# Autodesk Inventor assembly: Assy_all
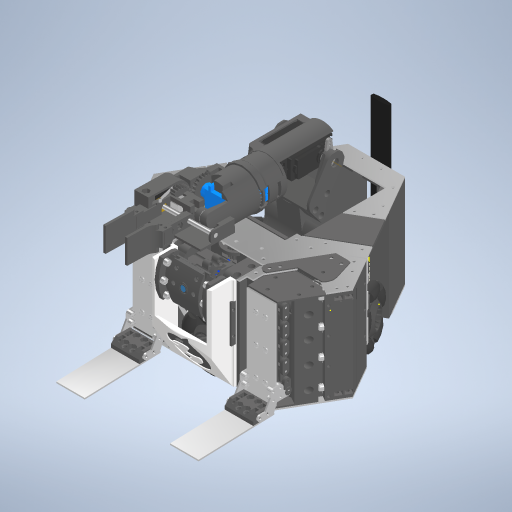
[picture p0: Inventor's stored thumbnail of the model, 512x512]
Saved by Autodesk Inventor 2024.1 (Build 281209000, 209)
## iProperties
Created: 2025-03-04
Part Number: Assy_all
Document SubType Name: Assembly
Designer: hibik
Author: hibik
## Documents named in this file (15)
- C:\Users\hibik\Documents\Robomech\RESCUE\ORCA\hard\Assy_all.iam
- C:\Users\hibik\Documents\Robomech\RESCUE\ORCA\hard\Assy_cam_connection.iam
- C:\Users\hibik\Documents\Robomech\RESCUE\ORCA\hard\flame_back\flame_back.ipt
- C:\Users\hibik\Documents\Robomech\RESCUE\ORCA\hard\board\core_power.iam
- C:\Users\hibik\Documents\Robomech\RESCUE\ORCA\hard\board\core_usp.iam
- C:\Users\hibik\Documents\Robomech\RESCUE\ORCA\hard\std_parts\battery.ipt
- C:\Users\hibik\Documents\Robomech\RESCUE\ORCA\hard\std_parts\emergency_button.ipt
- C:\Users\hibik\Documents\Robomech\RESCUE\ORCA\hard\flame_back\flame_upper_back.ipt
- C:\Users\hibik\Documents\Robomech\RESCUE\ORCA\hard\flame_back\flame_side_right.ipt
- C:\Users\hibik\Documents\Robomech\RESCUE\ORCA\hard\flame_back\flame_side_left.ipt
- C:\Users\hibik\Documents\Robomech\RESCUE\ORCA\hard\flame_back\battery_holder_spring.ipt
- C:\Users\hibik\Documents\Robomech\RESCUE\ORCA\hard\flame_back\battery_holder_cover.ipt
- C:\Users\hibik\Documents\Robomech\RESCUE\ORCA\hard\std_parts\Buffalo_Wl-U2-433DHP.ipt
- C:\Users\hibik\Documents\Robomech\RESCUE\ORCA\hard\flame_back\cover_setter_side_front.ipt
- C:\Users\hibik\Documents\Robomech\RESCUE\ORCA\hard\cover\Assy_cover_front.iam
## Components (15 placed, 14 different names)
1. Assy_cam_connection:1 [sub-assembly] — メイト:1, フラッシュ:1, フラッシュ:2, メイト:4, メイト:11, 挿入:7, 挿入:8, 挿入:9, 挿入:10, メイト:13, フラッシュ:10, メイト:14
2. flame_back:1 — メイト:1, フラッシュ:1, フラッシュ:2, 挿入:2, 挿入:3, メイト:2, フラッシュ:3, フラッシュ:4, メイト:5, メイト:6, メイト:8, フラッシュ:9, メイト:9, メイト:10, メイト:12
3. core_power:1 [sub-assembly] — 挿入:2, 挿入:3
4. battery:1 — メイト:10, メイト:11, メイト:12
5. core_usp:1 [sub-assembly] — 挿入:4, 挿入:5
6. emergency_button:1 — 挿入:6, 角度:1
7. flame_upper_back:1 — メイト:2, フラッシュ:3, フラッシュ:4, フラッシュ:5, フラッシュ:6, メイト:3, フラッシュ:7, フラッシュ:8, メイト:7
8. flame_side_right:1 — フラッシュ:5, フラッシュ:6, メイト:3, 挿入:4, 挿入:5
9. flame_side_left:1 — フラッシュ:7, フラッシュ:8, メイト:4, 挿入:6, 角度:1
10. battery_holder_spring:1 — メイト:5, メイト:6, メイト:7
11. battery_holder_cover:1 — メイト:8, フラッシュ:9, メイト:9
12. Buffalo_Wl-U2-433DHP:1
13. cover_setter_side_front:1 — 挿入:7, 挿入:8
14. cover_setter_side_front:2 — 挿入:9, 挿入:10
15. Assy_cover_front:1 [sub-assembly] — メイト:13, フラッシュ:10, メイト:14
## Relationships (34: Mate 14, Flush 10, Insert 9, Angle 1)
- メイト:1 [Mate]: Assy_cam_connection:1 ↔ flame_back:1
- フラッシュ:1 [Flush]: Assy_cam_connection:1 ↔ flame_back:1
- フラッシュ:2 [Flush]: Assy_cam_connection:1 ↔ flame_back:1
- 挿入:2 [Insert]: flame_back:1 ↔ core_power:1
- 挿入:3 [Insert]: flame_back:1 ↔ core_power:1
- メイト:2 [Mate]: flame_back:1 ↔ flame_upper_back:1
- フラッシュ:3 [Flush]: flame_back:1 ↔ flame_upper_back:1
- フラッシュ:4 [Flush]: flame_back:1 ↔ flame_upper_back:1
- フラッシュ:5 [Flush]: flame_upper_back:1 ↔ flame_side_right:1
- フラッシュ:6 [Flush]: flame_upper_back:1 ↔ flame_side_right:1
- メイト:3 [Mate] (1 mm): flame_upper_back:1 ↔ flame_side_right:1
- フラッシュ:7 [Flush]: flame_upper_back:1 ↔ flame_side_left:1
- フラッシュ:8 [Flush]: flame_upper_back:1 ↔ flame_side_left:1
- メイト:4 [Mate] (1 mm): Assy_cam_connection:1 ↔ flame_side_left:1
- 挿入:4 [Insert]: core_usp:1 ↔ flame_side_right:1
- 挿入:5 [Insert]: core_usp:1 ↔ flame_side_right:1
- 挿入:6 [Insert]: emergency_button:1 ↔ flame_side_left:1
- 角度:1 [Angle] (0 deg): emergency_button:1 ↔ flame_side_left:1
- メイト:5 [Mate] (0.25 mm): flame_back:1 ↔ battery_holder_spring:1
- メイト:6 [Mate] (0.25 mm): flame_back:1 ↔ battery_holder_spring:1
- メイト:7 [Mate]: flame_upper_back:1 ↔ battery_holder_spring:1
- メイト:8 [Mate]: flame_back:1 ↔ battery_holder_cover:1
- フラッシュ:9 [Flush]: flame_back:1 ↔ battery_holder_cover:1
- メイト:9 [Mate]: flame_back:1 ↔ battery_holder_cover:1
- メイト:10 [Mate]: flame_back:1 ↔ battery:1
- メイト:11 [Mate]: Assy_cam_connection:1 ↔ battery:1
- メイト:12 [Mate]: flame_back:1 ↔ battery:1
- 挿入:7 [Insert]: Assy_cam_connection:1 ↔ cover_setter_side_front:1
- 挿入:8 [Insert]: Assy_cam_connection:1 ↔ cover_setter_side_front:1
- 挿入:9 [Insert]: Assy_cam_connection:1 ↔ cover_setter_side_front:2
- 挿入:10 [Insert]: Assy_cam_connection:1 ↔ cover_setter_side_front:2
- メイト:13 [Mate]: Assy_cam_connection:1 ↔ Assy_cover_front:1
- フラッシュ:10 [Flush]: Assy_cam_connection:1 ↔ Assy_cover_front:1
- メイト:14 [Mate]: Assy_cam_connection:1 ↔ Assy_cover_front:1
